# Autodesk Inventor assembly: ASSEMBLY_Electromagnet
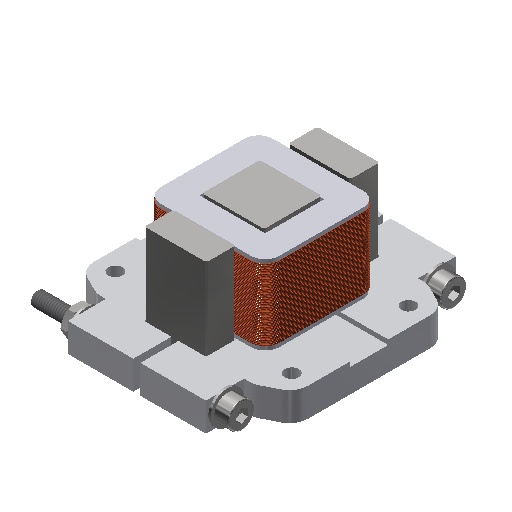
[picture p0: Inventor's stored thumbnail of the model, 512x512]
Saved by Autodesk Inventor 2025 (Build 290162010, 162A)
## iProperties
Created: 2018-05-26
Part Number: ASSEMBLY_Electromagnet
Document SubType Name: Assembly
Designer: Andrzej
Author: Andrzej
## Documents named in this file (8)
- D:\_ANDRZEJ_LACZEWSKI\_OTHER\MLTDIS - SMD parts bowl feeder prototype\MCAD\1_REV1\ASSEMBLY_MAIN_REVA\ASSEMBLY_Electromagnet.iam
- D:\_ANDRZEJ_LACZEWSKI\_OTHER\MLTDIS - SMD parts bowl feeder prototype\MCAD\1_REV1\__COTS_PARTS\COTS_GENERIC_Transformer_Electromagnet_Coil_Layer.ipt
- D:\_ANDRZEJ_LACZEWSKI\_OTHER\MLTDIS - SMD parts bowl feeder prototype\MCAD\1_REV1\__COTS_PARTS\COTS_GENERIC_Transformer_Core.ipt
- D:\_ANDRZEJ_LACZEWSKI\_OTHER\MLTDIS - SMD parts bowl feeder prototype\MCAD\1_REV1\ASSEMBLY_MAIN_REVA\3DP_ABS_Electromagnet_Clamps.ipt
- D:\_ANDRZEJ_LACZEWSKI\_OTHER\MLTDIS - SMD parts bowl feeder prototype\MCAD\1_REV1\ASSEMBLY_MAIN_REVA\3DP_ABS_Electromagnet_Coil_Holder.ipt
- D:\_ANDRZEJ_LACZEWSKI\_OTHER\MLTDIS - SMD parts bowl feeder prototype\MCAD\1_REV1\__CONTENT_CENTER_PARTS\en-US\DIN 125-2  A\DIN 125-2 - A 3,2A.ipt
- D:\_ANDRZEJ_LACZEWSKI\_OTHER\MLTDIS - SMD parts bowl feeder prototype\MCAD\1_REV1\__CONTENT_CENTER_PARTS\en-US\DIN 934\DIN 934 - M3 x 0,5.ipt
- D:\_ANDRZEJ_LACZEWSKI\_OTHER\MLTDIS - SMD parts bowl feeder prototype\MCAD\1_REV1\__COTS_PARTS\DIN 912 - M3 x 0,5 x 40 x 18.ipt
## Components (62 placed, 7 different names)
1. COTS_GENERIC_Transformer_Core:1 — Mate:1, Mate:2, Mate:3, Mate:4, Flush:1, Flush:2, Mate:11, Mate:12, Mate:13
2. 3DP_ABS_Electromagnet_Clamps:1 — Mate:1, Mate:4, Flush:1, Mate:14, Mate:15, Mate:16, Mate:17, Mate:18, Mate:20
3. 3DP_ABS_Electromagnet_Clamps:2 — Mate:2, Mate:3, Flush:2, Mate:19, Mate:21
4. 3DP_ABS_Electromagnet_Coil_Holder:1 — Mate:8, Mate:9, Mate:10, Mate:11, Mate:12, Mate:13
5. DIN 125-2 A A 3,2:1 — Mate:14, Mate:15, Insert:1
6. DIN 912 - replaced by DIN EN ISO 4762 M3 x 30:3 — Insert:1
7. DIN 125-2 A A 3,2:2 — Mate:18, Mate:19, Insert:3
8. DIN 934 - replaced by DIN EN 24032/28673/28674 M3:1 — Insert:3
9. DIN 125-2 A A 3,2:3 — Mate:16, Mate:17, Insert:2
10. DIN 912 - replaced by DIN EN ISO 4762 M3 x 30:2 — Insert:2
11. DIN 125-2 A A 3,2:4 — Mate:20, Mate:21, Insert:4
12. DIN 934 - replaced by DIN EN 24032/28673/28674 M3:2 — Insert:4
13. COTS_GENERIC_Transformer_Electromagnet_Coil_Layer:1 — Mate:8, Mate:9, Mate:10
14. COTS_GENERIC_Transformer_Electromagnet_Coil_Layer:2
15. COTS_GENERIC_Transformer_Electromagnet_Coil_Layer:3
16. COTS_GENERIC_Transformer_Electromagnet_Coil_Layer:4
17. COTS_GENERIC_Transformer_Electromagnet_Coil_Layer:5
18. COTS_GENERIC_Transformer_Electromagnet_Coil_Layer:6
19. COTS_GENERIC_Transformer_Electromagnet_Coil_Layer:7
20. COTS_GENERIC_Transformer_Electromagnet_Coil_Layer:8
21. COTS_GENERIC_Transformer_Electromagnet_Coil_Layer:9
22. COTS_GENERIC_Transformer_Electromagnet_Coil_Layer:10
23. COTS_GENERIC_Transformer_Electromagnet_Coil_Layer:11
24. COTS_GENERIC_Transformer_Electromagnet_Coil_Layer:12
25. COTS_GENERIC_Transformer_Electromagnet_Coil_Layer:13
26. COTS_GENERIC_Transformer_Electromagnet_Coil_Layer:14
27. COTS_GENERIC_Transformer_Electromagnet_Coil_Layer:15
28. COTS_GENERIC_Transformer_Electromagnet_Coil_Layer:16
29. COTS_GENERIC_Transformer_Electromagnet_Coil_Layer:17
30. COTS_GENERIC_Transformer_Electromagnet_Coil_Layer:18
31. COTS_GENERIC_Transformer_Electromagnet_Coil_Layer:19
32. COTS_GENERIC_Transformer_Electromagnet_Coil_Layer:20
33. COTS_GENERIC_Transformer_Electromagnet_Coil_Layer:21
34. COTS_GENERIC_Transformer_Electromagnet_Coil_Layer:22
35. COTS_GENERIC_Transformer_Electromagnet_Coil_Layer:23
36. COTS_GENERIC_Transformer_Electromagnet_Coil_Layer:24
37. COTS_GENERIC_Transformer_Electromagnet_Coil_Layer:25
38. COTS_GENERIC_Transformer_Electromagnet_Coil_Layer:26
39. COTS_GENERIC_Transformer_Electromagnet_Coil_Layer:27
40. COTS_GENERIC_Transformer_Electromagnet_Coil_Layer:28
41. COTS_GENERIC_Transformer_Electromagnet_Coil_Layer:29
42. COTS_GENERIC_Transformer_Electromagnet_Coil_Layer:30
43. COTS_GENERIC_Transformer_Electromagnet_Coil_Layer:31
44. COTS_GENERIC_Transformer_Electromagnet_Coil_Layer:32
45. COTS_GENERIC_Transformer_Electromagnet_Coil_Layer:33
46. COTS_GENERIC_Transformer_Electromagnet_Coil_Layer:34
47. COTS_GENERIC_Transformer_Electromagnet_Coil_Layer:35
48. COTS_GENERIC_Transformer_Electromagnet_Coil_Layer:36
49. COTS_GENERIC_Transformer_Electromagnet_Coil_Layer:37
50. COTS_GENERIC_Transformer_Electromagnet_Coil_Layer:38
51. COTS_GENERIC_Transformer_Electromagnet_Coil_Layer:39
52. COTS_GENERIC_Transformer_Electromagnet_Coil_Layer:40
53. COTS_GENERIC_Transformer_Electromagnet_Coil_Layer:41
54. COTS_GENERIC_Transformer_Electromagnet_Coil_Layer:42
55. COTS_GENERIC_Transformer_Electromagnet_Coil_Layer:43
56. COTS_GENERIC_Transformer_Electromagnet_Coil_Layer:44
57. COTS_GENERIC_Transformer_Electromagnet_Coil_Layer:45
58. COTS_GENERIC_Transformer_Electromagnet_Coil_Layer:46
59. COTS_GENERIC_Transformer_Electromagnet_Coil_Layer:47
60. COTS_GENERIC_Transformer_Electromagnet_Coil_Layer:48
61. COTS_GENERIC_Transformer_Electromagnet_Coil_Layer:49
62. COTS_GENERIC_Transformer_Electromagnet_Coil_Layer:50
## Component patterns: (50 elements, first: COTS_GENERIC_Transformer_Electromagnet_Coil_Layer:1)
## Relationships (24: Mate 18, Insert 4, Flush 2)
- Mate:1: COTS_GENERIC_Transformer_Core:1 ↔ 3DP_ABS_Electromagnet_Clamps:1
- Mate:2: COTS_GENERIC_Transformer_Core:1 ↔ 3DP_ABS_Electromagnet_Clamps:2
- Mate:3 (0.1 mm): COTS_GENERIC_Transformer_Core:1 ↔ 3DP_ABS_Electromagnet_Clamps:2
- Mate:4 (0.1 mm): COTS_GENERIC_Transformer_Core:1 ↔ 3DP_ABS_Electromagnet_Clamps:1
- Flush:1: COTS_GENERIC_Transformer_Core:1 ↔ 3DP_ABS_Electromagnet_Clamps:1
- Flush:2: COTS_GENERIC_Transformer_Core:1 ↔ 3DP_ABS_Electromagnet_Clamps:2
- Mate:8: 3DP_ABS_Electromagnet_Coil_Holder:1 ↔ COTS_GENERIC_Transformer_Electromagnet_Coil_Layer:1
- Mate:9: 3DP_ABS_Electromagnet_Coil_Holder:1 ↔ COTS_GENERIC_Transformer_Electromagnet_Coil_Layer:1
- Mate:10: 3DP_ABS_Electromagnet_Coil_Holder:1 ↔ COTS_GENERIC_Transformer_Electromagnet_Coil_Layer:1
- Mate:11: COTS_GENERIC_Transformer_Core:1 ↔ 3DP_ABS_Electromagnet_Coil_Holder:1
- Mate:12 (0.15 mm): COTS_GENERIC_Transformer_Core:1 ↔ 3DP_ABS_Electromagnet_Coil_Holder:1
- Mate:13 (0.375 mm): COTS_GENERIC_Transformer_Core:1 ↔ 3DP_ABS_Electromagnet_Coil_Holder:1
- Mate:14: 3DP_ABS_Electromagnet_Clamps:1 ↔ DIN 125-2 A A 3,2:1
- Mate:15: 3DP_ABS_Electromagnet_Clamps:1 ↔ DIN 125-2 A A 3,2:1
- Mate:16: 3DP_ABS_Electromagnet_Clamps:1 ↔ DIN 125-2 A A 3,2:3
- Mate:17: 3DP_ABS_Electromagnet_Clamps:1 ↔ DIN 125-2 A A 3,2:3
- Insert:1: DIN 125-2 A A 3,2:1 ↔ DIN 912 - replaced by DIN EN ISO 4762 M3 x 30:3
- Insert:2: DIN 125-2 A A 3,2:3 ↔ DIN 912 - replaced by DIN EN ISO 4762 M3 x 30:2
- Mate:18: 3DP_ABS_Electromagnet_Clamps:1 ↔ DIN 125-2 A A 3,2:2
- Mate:19: 3DP_ABS_Electromagnet_Clamps:2 ↔ DIN 125-2 A A 3,2:2
- Mate:20: 3DP_ABS_Electromagnet_Clamps:1 ↔ DIN 125-2 A A 3,2:4
- Mate:21: 3DP_ABS_Electromagnet_Clamps:2 ↔ DIN 125-2 A A 3,2:4
- Insert:3: DIN 125-2 A A 3,2:2 ↔ DIN 934 - replaced by DIN EN 24032/28673/28674 M3:1
- Insert:4: DIN 125-2 A A 3,2:4 ↔ DIN 934 - replaced by DIN EN 24032/28673/28674 M3:2
